# Autodesk Inventor assembly: Eplison gripper 1
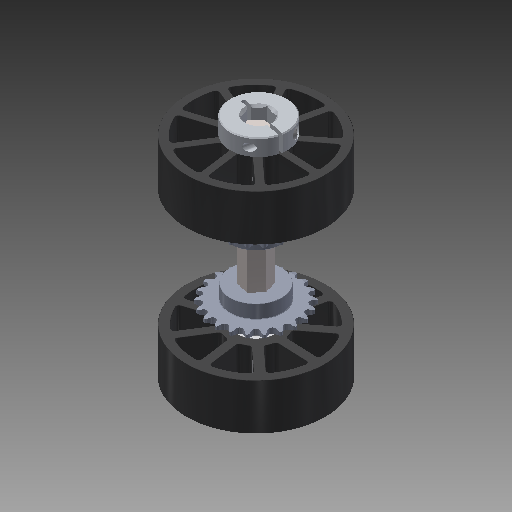
[picture p0: Inventor's stored thumbnail of the model, 512x512]
Saved by Autodesk Inventor 2019 (Build 230136000, 136)
## iProperties
Created: 2019-02-08
Part Number: Eplison gripper 1
Document SubType Name: Assembly
Designer: josh
Mass: 162.766 g
Surface Area: 809.446 cm^2
Volume: 162.766 cm^3
Density: 1 g/cm^3
Author: josh
## Documents named in this file (6)
- D:\Synthesis Robots\Epsilon\Epsilon Grabbers\Grabbing unit\Eplison gripper 1.iam
- D:\Synthesis Robots\Epsilon\Epsilon Grabbers\Grabbing unit\am-0856 500 Hex Shaft for Modulox REV3.ipt
- D:\Synthesis Robots\Epsilon\Epsilon Grabbers\am-0646 S25-22HA-500 Hex Sprocket.ipt
- D:\Synthesis Robots\Epsilon\Epsilon Grabbers\am-3946 3IN 500Hex Molded Compliant Wheel VER 2.ipt
- D:\Synthesis Robots\Epsilon\Epsilon Grabbers\am-0864 Hex Spacer for Modulox.ipt
- D:\Synthesis Robots\Epsilon\Epsilon Grabbers\am-1238 Collar Clamp, 0.5'' Hex Bore, Aluminum REV2.iam
## Components (9 placed, 5 different names)
1. am-0856 500 Hex Shaft for Modulox REV3:1 — Mate:18, Mate:19, Mate:21, Mate:22
2. am-0646 S25-22HA-500 Hex Sprocket:1
3. am-3946 3IN 500Hex Molded Compliant Wheel VER 2:1 — Mate:23
4. am-3946 3IN 500Hex Molded Compliant Wheel VER 2:2 — Mate:20
5. am-0646 S25-22HA-500 Hex Sprocket:2
6. am-0864 Hex Spacer for Modulox:1
7. am-0864 Hex Spacer for Modulox:2
8. am-1238 Collar Clamp, 0.5'' Hex Bore, Aluminum REV2:1 [sub-assembly] — Mate:18, Mate:19, Mate:20
9. am-1238 Collar Clamp, 0.5'' Hex Bore, Aluminum REV2:2 [sub-assembly] — Mate:21, Mate:22, Mate:23
## Relationships (23: Mate 23)
- [Mate]: am-0856 500 Hex Shaft for Modulox REV3:1 ↔ am-0646 S25-22HA-500 Hex Sprocket:1
- [Mate]: am-0856 500 Hex Shaft for Modulox REV3:1 ↔ am-0646 S25-22HA-500 Hex Sprocket:1
- [Mate]: am-0856 500 Hex Shaft for Modulox REV3:1 ↔ am-3946 3IN 500Hex Molded Compliant Wheel VER 2:1
- [Mate]: am-0856 500 Hex Shaft for Modulox REV3:1 ↔ am-3946 3IN 500Hex Molded Compliant Wheel VER 2:1
- [Mate]: am-0856 500 Hex Shaft for Modulox REV3:1 ↔ am-0646 S25-22HA-500 Hex Sprocket:2
- [Mate]: am-0856 500 Hex Shaft for Modulox REV3:1 ↔ am-0646 S25-22HA-500 Hex Sprocket:2
- [Mate]: am-0856 500 Hex Shaft for Modulox REV3:1 ↔ am-3946 3IN 500Hex Molded Compliant Wheel VER 2:2
- [Mate]: am-0856 500 Hex Shaft for Modulox REV3:1 ↔ am-3946 3IN 500Hex Molded Compliant Wheel VER 2:2
- [Mate]: am-0856 500 Hex Shaft for Modulox REV3:1 ↔ am-0864 Hex Spacer for Modulox:2
- [Mate]: am-0856 500 Hex Shaft for Modulox REV3:1 ↔ am-0864 Hex Spacer for Modulox:2
- [Mate]: am-0646 S25-22HA-500 Hex Sprocket:2 ↔ am-0864 Hex Spacer for Modulox:2
- [Mate]: am-3946 3IN 500Hex Molded Compliant Wheel VER 2:2 ↔ am-0864 Hex Spacer for Modulox:2
- [Mate]: am-0856 500 Hex Shaft for Modulox REV3:1 ↔ am-0864 Hex Spacer for Modulox:1
- [Mate]: am-0856 500 Hex Shaft for Modulox REV3:1 ↔ am-0864 Hex Spacer for Modulox:1
- [Mate]: am-0856 500 Hex Shaft for Modulox REV3:1 ↔ am-0864 Hex Spacer for Modulox:1
- [Mate]: am-0646 S25-22HA-500 Hex Sprocket:1 ↔ am-0864 Hex Spacer for Modulox:1
- [Mate]: am-3946 3IN 500Hex Molded Compliant Wheel VER 2:1 ↔ am-0864 Hex Spacer for Modulox:1
- Mate:18: am-0856 500 Hex Shaft for Modulox REV3:1 ↔ am-1238 Collar Clamp, 0.5'' Hex Bore, Aluminum REV2:1
- Mate:19: am-0856 500 Hex Shaft for Modulox REV3:1 ↔ am-1238 Collar Clamp, 0.5'' Hex Bore, Aluminum REV2:1
- Mate:20: am-3946 3IN 500Hex Molded Compliant Wheel VER 2:2 ↔ am-1238 Collar Clamp, 0.5'' Hex Bore, Aluminum REV2:1
- Mate:21: am-0856 500 Hex Shaft for Modulox REV3:1 ↔ am-1238 Collar Clamp, 0.5'' Hex Bore, Aluminum REV2:2
- Mate:22: am-0856 500 Hex Shaft for Modulox REV3:1 ↔ am-1238 Collar Clamp, 0.5'' Hex Bore, Aluminum REV2:2
- Mate:23: am-3946 3IN 500Hex Molded Compliant Wheel VER 2:1 ↔ am-1238 Collar Clamp, 0.5'' Hex Bore, Aluminum REV2:2
